# Autodesk Inventor assembly: 2f2
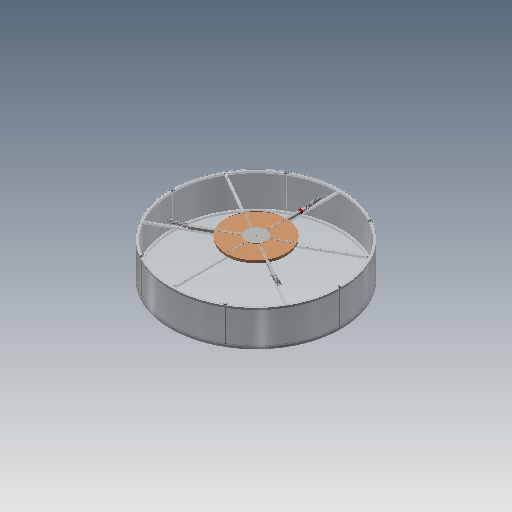
[picture p0: Inventor's stored thumbnail of the model, 512x512]
Saved by Autodesk Inventor 2017 (Build 210142000, 142)
## iProperties
Company: HERA Project
Created: 2013-06-27
Part Number: 2f2
Document SubType Name: Assembly
Designer: David DeBoer
Description: Feed backplane support assembly
Author: David DeBoer
Title: Feed backplane support
## Documents named in this file (6)
- C:\Users\krosie\Google Drive\HERA\hera-cad\feed\bpSupAssembly.iam
- C:\Users\krosie\Google Drive\HERA\hera-cad\feed\collar.ipt
- C:\Users\krosie\Google Drive\HERA\hera-cad\smallParts\D.ipt
- C:\Users\krosie\Google Drive\HERA\hera-cad\feed\bpMechSupAssembly.iam
- C:\Users\krosie\Google Drive\HERA\hera-cad\smallParts\spring.ipt
- C:\Users\krosie\Google Drive\HERA\hera-cad\feed\bpSupAssy37\bpSupAssy37.iam
## Components (9 placed, 5 different names)
1. bpMechSupAssembly:1 [sub-assembly] — Insert:11, Angle:1, Insert:19, Flush:2, Mate:1, Mate:2
2. collar:1 — Insert:19
3. bpSupAssy37:1 [sub-assembly] — Flush:2, Mate:1, Mate:2
4. D:1 — Insert:11, Insert:18
5. spring:1 — Insert:18, Angle:1
6. D:2
7. spring:2
8. D:3
9. spring:3
## Component patterns: (3 elements, first: D:1 + spring:1)
## Relationships (13: Mate 5, Insert 3, Tangent 3, Angle 1, Flush 1)
- Insert:11 (-35.56 mm): bpMechSupAssembly:1 ↔ D:1
- Insert:18: D:1 ↔ spring:1
- Angle:1 (190 deg): bpMechSupAssembly:1 ↔ spring:1
- Insert:19: bpMechSupAssembly:1 ↔ collar:1
- Flush:2: bpMechSupAssembly:1 ↔ bpSupAssy37:1
- Mate:1: bpMechSupAssembly:1 ↔ bpSupAssy37:1
- Mate:2: bpMechSupAssembly:1 ↔ bpSupAssy37:1
- [Mate]: collar:1 ↔ bpSupAssy37:1
- [Tangent]: collar:1 ↔ bpSupAssy37:1
- [Mate]: collar:1 ↔ bpSupAssy37:1
- [Tangent]: collar:1 ↔ bpSupAssy37:1
- [Mate]: collar:1 ↔ bpSupAssy37:1
- [Tangent]: collar:1 ↔ bpSupAssy37:1
